# Autodesk Inventor assembly: Rack-Rom
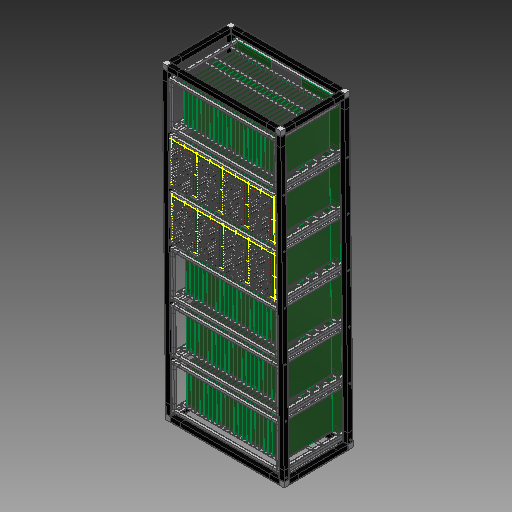
[picture p0: Inventor's stored thumbnail of the model, 512x512]
Saved by Autodesk Inventor 2018 (Build 220112000, 112)
## iProperties
Created: 2025-02-17
Part Number: Rack-Rom
Material: Všeobecné
Document SubType Name: Assembly
Designer: Jozko Mrkvicka
Author: Jozko Mrkvicka
## Documents named in this file (11)
- D:\05_Projekty\Projects_Inventor\Haluska9000\Rack-Rom.iam
- D:\05_Projekty\Projects_Inventor\Haluska9000\Profile-Connector\Profile-Connector#30x30xCorner.ipt
- D:\05_Projekty\Projects_Inventor\Haluska9000\Profile-Connector.ipt
- D:\05_Projekty\Projects_Inventor\Haluska9000\Profile-Square-Black.ipt
- D:\05_Projekty\Projects_Inventor\Haluska9000\Profile-T.ipt
- D:\05_Projekty\Projects_Inventor\Haluska9000\Profile-T\Profile-T#Rack-Rom.ipt
- D:\05_Projekty\Projects_Inventor\Haluska9000\Profile-Square-Black\Profile-Square#Rack-Rom-Length.ipt
- D:\05_Projekty\Projects_Inventor\Haluska9000\Profile-Square-Black\Profile-Square#Rack-Rom-Width.ipt
- D:\05_Projekty\Projects_Inventor\Haluska9000\Profile-Square-Black\Profile-Square#Rack-Rom-Height.ipt
- D:\05_Projekty\Projects_Inventor\Haluska9000\Cabinet-LogicCircuit.iam
- D:\05_Projekty\Projects_Inventor\Haluska9000\Panel-Mprom.iam
## Components (46 placed, 7 different names)
1. Profile-Connector#30x30xCorner:11 — Proti sobě:560, Proti sobě:561, Proti sobě:562, Proti sobě:572, Proti sobě:573, Proti sobě:574, Proti sobě:590, Proti sobě:591, Proti sobě:592
2. Profile-Connector#30x30xCorner:12 — Proti sobě:569, Proti sobě:570, Proti sobě:571, Proti sobě:575, Proti sobě:576, Proti sobě:577
3. Profile-Connector#30x30xCorner:13 — Proti sobě:581, Proti sobě:582, Proti sobě:583, Proti sobě:587, Proti sobě:588, Proti sobě:589
4. Profile-Connector#30x30xCorner:14 — Proti sobě:578, Proti sobě:579, Proti sobě:580, Proti sobě:584, Proti sobě:585, Proti sobě:586, Proti sobě:646, Proti sobě:647, Proti sobě:648
5. Profile-Square#Rack-Rom-Height:1 — Proti sobě:560, Proti sobě:561, Proti sobě:562, Proti sobě:581, Proti sobě:582, Proti sobě:583, Proti sobě:624, Stejný směr:36, Proti sobě:625, Stejný směr:40, Proti sobě:639, Proti sobě:640, Stejný směr:45, Stejný směr:46
6. Profile-Square#Rack-Rom-Height:3 — Proti sobě:569, Proti sobě:570, Proti sobě:571, Proti sobě:578, Proti sobě:579, Proti sobě:580, Proti sobě:623, Stejný směr:35, Proti sobě:626, Stejný směr:39, Proti sobě:629, Proti sobě:630, Proti sobě:637, Proti sobě:638, Stejný směr:43, Stejný směr:44, Proti sobě:641, Proti sobě:642
7. Profile-Square#Rack-Rom-Length:5 — Proti sobě:572, Proti sobě:573, Proti sobě:574, Proti sobě:620, Proti sobě:621, Proti sobě:622
8. Profile-Square#Rack-Rom-Length:6 — Proti sobě:575, Proti sobě:576, Proti sobě:577
9. Profile-Square#Rack-Rom-Length:11
10. Profile-Square#Rack-Rom-Length:12 — Proti sobě:646, Proti sobě:647, Proti sobě:648
11. Profile-Square#Rack-Rom-Width:7 — Proti sobě:584, Proti sobě:585, Proti sobě:586, Proti sobě:587, Proti sobě:588, Proti sobě:589
12. Profile-Square#Rack-Rom-Width:8 — Proti sobě:590, Proti sobě:591, Proti sobě:592
13. Profile-Square#Rack-Rom-Width:13
14. Profile-Square#Rack-Rom-Width:14 — Proti sobě:643, Proti sobě:644, Proti sobě:645
15. Profile-Connector#30x30xCorner:15
16. Profile-Connector#30x30xCorner:16 — Proti sobě:643, Proti sobě:644, Proti sobě:645
17. Profile-Connector#30x30xCorner:17 — Proti sobě:620, Proti sobě:621, Proti sobě:622, Proti sobě:631, Proti sobě:632, Proti sobě:633
18. Profile-Connector#30x30xCorner:18 — Proti sobě:634, Proti sobě:635, Proti sobě:636
19. Profile-T#Rack-Rom:1 — Proti sobě:623, Stejný směr:35, Stejný směr:37, Proti sobě:629
20. Profile-T#Rack-Rom:2 — Proti sobě:624, Stejný směr:36, Stejný směr:37, Proti sobě:649, Proti sobě:650
21. Profile-T#Rack-Rom:3 — Proti sobě:626, Stejný směr:39, Proti sobě:630
22. Profile-T#Rack-Rom:4 — Proti sobě:625, Stejný směr:40, Proti sobě:657
23. Profile-Square#Rack-Rom-Height:15 — Proti sobě:631, Proti sobě:632, Proti sobě:633, Proti sobě:653, Proti sobě:654, Stejný směr:49, Stejný směr:50
24. Profile-Square#Rack-Rom-Height:16 — Proti sobě:634, Proti sobě:635, Proti sobě:636, Proti sobě:651, Proti sobě:652, Stejný směr:51, Stejný směr:52, Proti sobě:655, Proti sobě:656
25. Profile-T#Rack-Rom:5 — Proti sobě:638, Stejný směr:43, Proti sobě:641
26. Profile-T#Rack-Rom:6 — Proti sobě:640, Stejný směr:46, Proti sobě:658
27. Profile-T#Rack-Rom:7 — Proti sobě:637, Stejný směr:44, Proti sobě:642
28. Profile-T#Rack-Rom:8 — Proti sobě:639, Stejný směr:45, Proti sobě:659
29. Cabinet-LogicCircuit:1 [sub-assembly] — Proti sobě:649, Proti sobě:650, Stejný směr:53, Stejný směr:58
30. Profile-T#Rack-Rom:9 — Proti sobě:651, Stejný směr:52, Proti sobě:655
31. Profile-T#Rack-Rom:10 — Proti sobě:654, Stejný směr:49, Proti sobě:660
32. Profile-T#Rack-Rom:11 — Proti sobě:652, Stejný směr:51, Proti sobě:656
33. Profile-T#Rack-Rom:12 — Proti sobě:653, Stejný směr:50, Proti sobě:661
34. Cabinet-LogicCircuit:2 [sub-assembly] — Stejný směr:53, Stejný směr:54, Stejný směr:58, Stejný směr:59, Proti sobě:657
35. Cabinet-LogicCircuit:3 [sub-assembly] — Stejný směr:54, Stejný směr:55, Stejný směr:59, Stejný směr:60, Proti sobě:658
36. Cabinet-LogicCircuit:4 [sub-assembly] — Stejný směr:55, Stejný směr:56, Stejný směr:60, Stejný směr:61, Proti sobě:659, Proti sobě:662, Stejný směr:63
37. Cabinet-LogicCircuit:5 [sub-assembly] — Stejný směr:56, Stejný směr:57, Stejný směr:61, Stejný směr:62, Proti sobě:660, Proti sobě:669, Stejný směr:77
38. Cabinet-LogicCircuit:6 [sub-assembly] — Stejný směr:57, Stejný směr:62, Proti sobě:661
39. Panel-Mprom:1 [sub-assembly] — Proti sobě:662, Stejný směr:63, Stejný směr:64, Proti sobě:663, Stejný směr:67
40. Panel-Mprom:2 [sub-assembly] — Stejný směr:66, Stejný směr:69, Proti sobě:664, Stejný směr:76
41. Panel-Mprom:3 [sub-assembly] — Stejný směr:65, Stejný směr:66, Stejný směr:68, Stejný směr:69, Proti sobě:664, Proti sobě:665
42. Panel-Mprom:4 [sub-assembly] — Stejný směr:64, Stejný směr:65, Proti sobě:663, Stejný směr:67, Stejný směr:68, Proti sobě:665
43. Panel-Mprom:5 [sub-assembly] — Proti sobě:669, Stejný směr:77
44. Panel-Mprom:6 [sub-assembly] — Stejný směr:76
45. Panel-Mprom:7 [sub-assembly]
46. Panel-Mprom:8 [sub-assembly]
## Relationships (133: Mate 90, Flush 43)
- Proti sobě:560 [Mate]: Profile-Connector#30x30xCorner:11 ↔ Profile-Square#Rack-Rom-Height:1
- Proti sobě:561 [Mate]: Profile-Connector#30x30xCorner:11 ↔ Profile-Square#Rack-Rom-Height:1
- Proti sobě:562 [Mate]: Profile-Connector#30x30xCorner:11 ↔ Profile-Square#Rack-Rom-Height:1
- Proti sobě:569 [Mate]: Profile-Connector#30x30xCorner:12 ↔ Profile-Square#Rack-Rom-Height:3
- Proti sobě:570 [Mate]: Profile-Connector#30x30xCorner:12 ↔ Profile-Square#Rack-Rom-Height:3
- Proti sobě:571 [Mate]: Profile-Connector#30x30xCorner:12 ↔ Profile-Square#Rack-Rom-Height:3
- Proti sobě:572 [Mate]: Profile-Connector#30x30xCorner:11 ↔ Profile-Square#Rack-Rom-Length:5
- Proti sobě:573 [Mate]: Profile-Connector#30x30xCorner:11 ↔ Profile-Square#Rack-Rom-Length:5
- Proti sobě:574 [Mate]: Profile-Connector#30x30xCorner:11 ↔ Profile-Square#Rack-Rom-Length:5
- Proti sobě:575 [Mate]: Profile-Connector#30x30xCorner:12 ↔ Profile-Square#Rack-Rom-Length:6
- Proti sobě:576 [Mate]: Profile-Connector#30x30xCorner:12 ↔ Profile-Square#Rack-Rom-Length:6
- Proti sobě:577 [Mate]: Profile-Connector#30x30xCorner:12 ↔ Profile-Square#Rack-Rom-Length:6
- Proti sobě:578 [Mate]: Profile-Connector#30x30xCorner:14 ↔ Profile-Square#Rack-Rom-Height:3
- Proti sobě:579 [Mate]: Profile-Connector#30x30xCorner:14 ↔ Profile-Square#Rack-Rom-Height:3
- Proti sobě:580 [Mate]: Profile-Connector#30x30xCorner:14 ↔ Profile-Square#Rack-Rom-Height:3
- Proti sobě:581 [Mate]: Profile-Connector#30x30xCorner:13 ↔ Profile-Square#Rack-Rom-Height:1
- Proti sobě:582 [Mate]: Profile-Connector#30x30xCorner:13 ↔ Profile-Square#Rack-Rom-Height:1
- Proti sobě:583 [Mate]: Profile-Connector#30x30xCorner:13 ↔ Profile-Square#Rack-Rom-Height:1
- Proti sobě:584 [Mate]: Profile-Connector#30x30xCorner:14 ↔ Profile-Square#Rack-Rom-Width:7
- Proti sobě:585 [Mate]: Profile-Connector#30x30xCorner:14 ↔ Profile-Square#Rack-Rom-Width:7
- Proti sobě:586 [Mate]: Profile-Connector#30x30xCorner:14 ↔ Profile-Square#Rack-Rom-Width:7
- Proti sobě:587 [Mate]: Profile-Connector#30x30xCorner:13 ↔ Profile-Square#Rack-Rom-Width:7
- Proti sobě:588 [Mate]: Profile-Connector#30x30xCorner:13 ↔ Profile-Square#Rack-Rom-Width:7
- Proti sobě:589 [Mate]: Profile-Connector#30x30xCorner:13 ↔ Profile-Square#Rack-Rom-Width:7
- Proti sobě:590 [Mate]: Profile-Connector#30x30xCorner:11 ↔ Profile-Square#Rack-Rom-Width:8
- Proti sobě:591 [Mate]: Profile-Connector#30x30xCorner:11 ↔ Profile-Square#Rack-Rom-Width:8
- Proti sobě:592 [Mate]: Profile-Connector#30x30xCorner:11 ↔ Profile-Square#Rack-Rom-Width:8
- [Mate]: Profile-Square#Rack-Rom-Length:11 ↔ Profile-Connector#30x30xCorner:15
- [Mate]: Profile-Square#Rack-Rom-Length:11 ↔ Profile-Connector#30x30xCorner:15
- [Mate]: Profile-Square#Rack-Rom-Length:11 ↔ Profile-Connector#30x30xCorner:15
- [Mate]: Profile-Square#Rack-Rom-Length:12 ↔ Profile-Connector#30x30xCorner:16
- [Mate]: Profile-Square#Rack-Rom-Length:12 ↔ Profile-Connector#30x30xCorner:16
- [Mate]: Profile-Square#Rack-Rom-Length:12 ↔ Profile-Connector#30x30xCorner:16
- [Mate]: Profile-Square#Rack-Rom-Width:13 ↔ Profile-Connector#30x30xCorner:18
- [Mate]: Profile-Square#Rack-Rom-Width:13 ↔ Profile-Connector#30x30xCorner:18
- [Mate]: Profile-Square#Rack-Rom-Width:13 ↔ Profile-Connector#30x30xCorner:18
- [Mate]: Profile-Square#Rack-Rom-Width:13 ↔ Profile-Connector#30x30xCorner:17
- [Mate]: Profile-Square#Rack-Rom-Width:13 ↔ Profile-Connector#30x30xCorner:17
- [Mate]: Profile-Square#Rack-Rom-Width:13 ↔ Profile-Connector#30x30xCorner:17
- [Mate]: Profile-Square#Rack-Rom-Width:14 ↔ Profile-Connector#30x30xCorner:15
- [Mate]: Profile-Square#Rack-Rom-Width:14 ↔ Profile-Connector#30x30xCorner:15
- [Mate]: Profile-Square#Rack-Rom-Width:14 ↔ Profile-Connector#30x30xCorner:15
- Proti sobě:620 [Mate]: Profile-Square#Rack-Rom-Length:5 ↔ Profile-Connector#30x30xCorner:17
- Proti sobě:621 [Mate]: Profile-Square#Rack-Rom-Length:5 ↔ Profile-Connector#30x30xCorner:17
- Proti sobě:622 [Mate]: Profile-Square#Rack-Rom-Length:5 ↔ Profile-Connector#30x30xCorner:17
- Proti sobě:623 [Mate]: Profile-Square#Rack-Rom-Height:3 ↔ Profile-T#Rack-Rom:1
- Stejný směr:35 [Flush]: Profile-Square#Rack-Rom-Height:3 ↔ Profile-T#Rack-Rom:1
- Proti sobě:624 [Mate]: Profile-Square#Rack-Rom-Height:1 ↔ Profile-T#Rack-Rom:2
- Stejný směr:36 [Flush]: Profile-Square#Rack-Rom-Height:1 ↔ Profile-T#Rack-Rom:2
- Stejný směr:37 [Flush]: Profile-T#Rack-Rom:1 ↔ Profile-T#Rack-Rom:2
- [Flush]: Profile-T#Rack-Rom:3 ↔ Profile-T#Rack-Rom:4
- Proti sobě:625 [Mate]: Profile-Square#Rack-Rom-Height:1 ↔ Profile-T#Rack-Rom:4
- Proti sobě:626 [Mate]: Profile-Square#Rack-Rom-Height:3 ↔ Profile-T#Rack-Rom:3
- Stejný směr:39 [Flush]: Profile-Square#Rack-Rom-Height:3 ↔ Profile-T#Rack-Rom:3
- Stejný směr:40 [Flush]: Profile-Square#Rack-Rom-Height:1 ↔ Profile-T#Rack-Rom:4
- Proti sobě:629 [Mate]: Profile-Square#Rack-Rom-Height:3 ↔ Profile-T#Rack-Rom:1
- Proti sobě:630 [Mate]: Profile-Square#Rack-Rom-Height:3 ↔ Profile-T#Rack-Rom:3
- Proti sobě:631 [Mate]: Profile-Connector#30x30xCorner:17 ↔ Profile-Square#Rack-Rom-Height:15
- Proti sobě:632 [Mate]: Profile-Connector#30x30xCorner:17 ↔ Profile-Square#Rack-Rom-Height:15
- Proti sobě:633 [Mate]: Profile-Connector#30x30xCorner:17 ↔ Profile-Square#Rack-Rom-Height:15
- Proti sobě:634 [Mate]: Profile-Connector#30x30xCorner:18 ↔ Profile-Square#Rack-Rom-Height:16
- Proti sobě:635 [Mate]: Profile-Connector#30x30xCorner:18 ↔ Profile-Square#Rack-Rom-Height:16
- Proti sobě:636 [Mate]: Profile-Connector#30x30xCorner:18 ↔ Profile-Square#Rack-Rom-Height:16
- [Flush]: Profile-T#Rack-Rom:5 ↔ Profile-T#Rack-Rom:6
- [Flush]: Profile-T#Rack-Rom:7 ↔ Profile-T#Rack-Rom:8
- Proti sobě:637 [Mate]: Profile-Square#Rack-Rom-Height:3 ↔ Profile-T#Rack-Rom:7
- Proti sobě:638 [Mate]: Profile-Square#Rack-Rom-Height:3 ↔ Profile-T#Rack-Rom:5
- Proti sobě:639 [Mate]: Profile-Square#Rack-Rom-Height:1 ↔ Profile-T#Rack-Rom:8
- Proti sobě:640 [Mate]: Profile-Square#Rack-Rom-Height:1 ↔ Profile-T#Rack-Rom:6
- Stejný směr:43 [Flush]: Profile-Square#Rack-Rom-Height:3 ↔ Profile-T#Rack-Rom:5
- Stejný směr:44 [Flush]: Profile-Square#Rack-Rom-Height:3 ↔ Profile-T#Rack-Rom:7
- Stejný směr:45 [Flush]: Profile-Square#Rack-Rom-Height:1 ↔ Profile-T#Rack-Rom:8
- Stejný směr:46 [Flush]: Profile-Square#Rack-Rom-Height:1 ↔ Profile-T#Rack-Rom:6
- Proti sobě:641 [Mate]: Profile-Square#Rack-Rom-Height:3 ↔ Profile-T#Rack-Rom:5
- Proti sobě:642 [Mate]: Profile-Square#Rack-Rom-Height:3 ↔ Profile-T#Rack-Rom:7
- Proti sobě:643 [Mate]: Profile-Square#Rack-Rom-Width:14 ↔ Profile-Connector#30x30xCorner:16
- Proti sobě:644 [Mate]: Profile-Square#Rack-Rom-Width:14 ↔ Profile-Connector#30x30xCorner:16
- Proti sobě:645 [Mate]: Profile-Square#Rack-Rom-Width:14 ↔ Profile-Connector#30x30xCorner:16
- Proti sobě:646 [Mate]: Profile-Connector#30x30xCorner:14 ↔ Profile-Square#Rack-Rom-Length:12
- Proti sobě:647 [Mate]: Profile-Connector#30x30xCorner:14 ↔ Profile-Square#Rack-Rom-Length:12
- Proti sobě:648 [Mate]: Profile-Connector#30x30xCorner:14 ↔ Profile-Square#Rack-Rom-Length:12
- Proti sobě:649 [Mate]: Profile-T#Rack-Rom:2 ↔ Cabinet-LogicCircuit:1
- Proti sobě:650 [Mate] (1 mm): Profile-T#Rack-Rom:2 ↔ Cabinet-LogicCircuit:1
- [Flush]: Profile-T#Rack-Rom:9 ↔ Profile-T#Rack-Rom:10
- [Flush]: Profile-T#Rack-Rom:11 ↔ Profile-T#Rack-Rom:12
- Proti sobě:651 [Mate]: Profile-Square#Rack-Rom-Height:16 ↔ Profile-T#Rack-Rom:9
- Proti sobě:652 [Mate]: Profile-Square#Rack-Rom-Height:16 ↔ Profile-T#Rack-Rom:11
- Proti sobě:653 [Mate]: Profile-Square#Rack-Rom-Height:15 ↔ Profile-T#Rack-Rom:12
- Proti sobě:654 [Mate]: Profile-Square#Rack-Rom-Height:15 ↔ Profile-T#Rack-Rom:10
- Stejný směr:49 [Flush]: Profile-Square#Rack-Rom-Height:15 ↔ Profile-T#Rack-Rom:10
- Stejný směr:50 [Flush]: Profile-Square#Rack-Rom-Height:15 ↔ Profile-T#Rack-Rom:12
- Stejný směr:51 [Flush]: Profile-Square#Rack-Rom-Height:16 ↔ Profile-T#Rack-Rom:11
- Stejný směr:52 [Flush]: Profile-Square#Rack-Rom-Height:16 ↔ Profile-T#Rack-Rom:9
- Proti sobě:655 [Mate]: Profile-Square#Rack-Rom-Height:16 ↔ Profile-T#Rack-Rom:9
- Proti sobě:656 [Mate]: Profile-Square#Rack-Rom-Height:16 ↔ Profile-T#Rack-Rom:11
- Stejný směr:53 [Flush]: Cabinet-LogicCircuit:1 ↔ Cabinet-LogicCircuit:2
- Stejný směr:54 [Flush]: Cabinet-LogicCircuit:2 ↔ Cabinet-LogicCircuit:3
- Stejný směr:55 [Flush]: Cabinet-LogicCircuit:3 ↔ Cabinet-LogicCircuit:4
- Stejný směr:56 [Flush]: Cabinet-LogicCircuit:4 ↔ Cabinet-LogicCircuit:5
- Stejný směr:57 [Flush]: Cabinet-LogicCircuit:5 ↔ Cabinet-LogicCircuit:6
- Stejný směr:58 [Flush]: Cabinet-LogicCircuit:1 ↔ Cabinet-LogicCircuit:2
- Stejný směr:59 [Flush]: Cabinet-LogicCircuit:2 ↔ Cabinet-LogicCircuit:3
- Stejný směr:60 [Flush]: Cabinet-LogicCircuit:3 ↔ Cabinet-LogicCircuit:4
- Stejný směr:61 [Flush]: Cabinet-LogicCircuit:4 ↔ Cabinet-LogicCircuit:5
- Stejný směr:62 [Flush]: Cabinet-LogicCircuit:5 ↔ Cabinet-LogicCircuit:6
- Proti sobě:657 [Mate]: Profile-T#Rack-Rom:4 ↔ Cabinet-LogicCircuit:2
- Proti sobě:658 [Mate]: Profile-T#Rack-Rom:6 ↔ Cabinet-LogicCircuit:3
- Proti sobě:659 [Mate]: Profile-T#Rack-Rom:8 ↔ Cabinet-LogicCircuit:4
- Proti sobě:660 [Mate]: Profile-T#Rack-Rom:10 ↔ Cabinet-LogicCircuit:5
- Proti sobě:661 [Mate]: Profile-T#Rack-Rom:12 ↔ Cabinet-LogicCircuit:6
- Proti sobě:662 [Mate]: Cabinet-LogicCircuit:4 ↔ Panel-Mprom:1
- Stejný směr:63 [Flush] (-15 mm): Cabinet-LogicCircuit:4 ↔ Panel-Mprom:1
- Stejný směr:64 [Flush]: Panel-Mprom:1 ↔ Panel-Mprom:4
- Stejný směr:65 [Flush]: Panel-Mprom:3 ↔ Panel-Mprom:4
- Stejný směr:66 [Flush]: Panel-Mprom:2 ↔ Panel-Mprom:3
- Proti sobě:663 [Mate]: Panel-Mprom:1 ↔ Panel-Mprom:4
- Stejný směr:67 [Flush]: Panel-Mprom:1 ↔ Panel-Mprom:4
- Stejný směr:68 [Flush]: Panel-Mprom:3 ↔ Panel-Mprom:4
- Stejný směr:69 [Flush]: Panel-Mprom:2 ↔ Panel-Mprom:3
- Proti sobě:664 [Mate]: Panel-Mprom:2 ↔ Panel-Mprom:3
- Proti sobě:665 [Mate]: Panel-Mprom:3 ↔ Panel-Mprom:4
- [Flush]: Panel-Mprom:5 ↔ Panel-Mprom:8
- [Flush]: Panel-Mprom:7 ↔ Panel-Mprom:8
- [Flush]: Panel-Mprom:6 ↔ Panel-Mprom:7
- [Mate]: Panel-Mprom:5 ↔ Panel-Mprom:8
- [Flush]: Panel-Mprom:5 ↔ Panel-Mprom:8
- [Flush]: Panel-Mprom:7 ↔ Panel-Mprom:8
- [Flush]: Panel-Mprom:6 ↔ Panel-Mprom:7
- [Mate]: Panel-Mprom:6 ↔ Panel-Mprom:7
- [Mate]: Panel-Mprom:7 ↔ Panel-Mprom:8
- Proti sobě:669 [Mate]: Cabinet-LogicCircuit:5 ↔ Panel-Mprom:5
- Stejný směr:76 [Flush]: Panel-Mprom:2 ↔ Panel-Mprom:6
- Stejný směr:77 [Flush] (15 mm): Cabinet-LogicCircuit:5 ↔ Panel-Mprom:5
## Named parameters: d1044_d1033 = 0 mm, d1045_d1034 = 0 mm, d1046_d1035 = 0 mm, d1047_d1036 = 0 mm, d1048_d1037 = 0 mm, d1049_d1038 = 0 mm, d1050_d1039 = 0 mm, d1051_d1040 = 0 mm, d1052_d1041 = 0 mm, d1059_d1021 = 0 mm, d1060_d1022 = 0 mm, d1061_d1023 = 0 mm, d1062_d1024 = 0 mm, d1063_d1025 = 0 mm, d1064_d1026 = 0 mm, d1077_d1076 = 0 mm, d1092_d1077_d1076 = 0 mm, d1093_d1077_d1076 = 0 mm, d1123_d1093_d1077_d1076 = 0 mm, d1124_d1093_d1077_d1076 = 0 mm, d1161_d1152 = 0 mm, d1162_d1153 = 0 mm, d1163_d1154 = 0 mm, d1164_d1155 = 0 mm, d1165_d1156 = 0 mm, d1166_d1157 = 0 mm, d1167_d1158 = 0 mm, d1168_d1159 = 0 mm, d1169_d1160 = 0 mm
